# Autodesk Inventor assembly: CPRC16-6-6
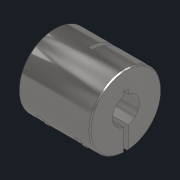
[picture p0: Inventor's stored thumbnail of the model, 180x180]
Saved by Autodesk Inventor 2022 (Build 260153000, 153)
## iProperties
Category: PARTsolutions
Company: MISUMI
Part Number: CPRC16-6-6
Catalog Web Link: www.cadenas.de
Description: CPRC, CPRSC-Couplings - Rigid - Clamping Type
Vendor: MISUMI
Document SubType Name: Assembly
Designer: partserver
Manufacturer: MISUMI
Mass: 2.52025 g
Surface Area: 21.4845 cm^2
Volume: 2.52025 cm^3
Density: 1 g/cm^3
PSOL_IDENT_0: {$CADENAS_DATA\23d-libs\misumi\metric\50_couplings\cprc_asmtab.prj},181 {VTYP=3D},{STYP=ASSTAB},{NB=
PSOL_IDENT_1: CPRC16-6-6},{LINA=CPRC16-6-6},{NN=CPRC, CPRSC},{DATE=30.06.2021 13:24:31},{GEOMDATE=17.01.2008},{VER
PSOL_IDENT_2: SION=},{LINEID=10},{WBVAR=MAT,DD1,DD2},{WBNUMERIC=}  {NB=CPRC16-6-6},{LINA=CPRC16-6-6},{KT=DUMMY},{P
PSOL_IDENT_3: N=CPRC16-6-6},{MAT=1},{MATALG='1','Aluminum Alloy','2','Stainless Steel'},{ST=Alumite},{AC=Hexagon S
PSOL_IDENT_4: ocket Head Cap Screws},{TYPE=CPRC},{D=16},{DD1=6},{DD1ALG1='5','5','6','6'},{DL=6},{DD2=6},{DD2ALG1='
PSOL_IDENT_5: 6','6'},{DR=6},{L=16},{M=2.5},{TSI=M2.5},{A=5},{A1=5.000},{TT=1},{TT1=1.000},{F=3.75},{T=1},{AT=0.3}
PSOL_IDENT_6: ,{F1=3.750},{TSI1=4.800},{SC1=2.500},{SC2=5.970},{TSMD=2.500},{TSMIN=2.013},{L6=4.000},{PPATH=cprc_t
PSOL_IDENT_7: emp.prj}
NB: CPRC16-6-6
NN: CPRC, CPRSC
NT: Couplings - Rigid - Clamping Type
NBSYN: $TYPE.$D.-$DD1.-$DD2.
LINA: CPRC16-6-6
CATALOG: Misumi
PN: CPRC16-6-6
MAT: Aluminum Alloy
ST: Clear Anodizing
AC: Hexagon Socket Head Cap Screws
D: 16
DD1: 6
DD2: 6
L: 16
M: 2.5
A: 5
TT: 1
F: 3.75
T: 1
SUPPLIER: MISUMI
ARTICLENO: CPRC16-6-6
BOMINFO: CPRC16-6-6
CREATOR: CADENAS GmbH
Title: CPRC16-6-6
Author: Cadenas PARTsolutions
Comments: Couplings - Rigid - Clamping Type
## Documents named in this file (3)
- C:\Users\yuta0\Downloads\0928\CPRC16-6-6.iam
- C:\Users\yuta0\Downloads\0928\D_CPRC16-6-6.ipt
- C:\Users\yuta0\Downloads\0928\M2_5.ipt
## Components (3 placed, 2 different names)
1. D_CPRC16-6-6:1 — L_XY@1 <-> SCW_XY@2, L_Z@1 <-> SCW_Z@2, L_YZ@1 <-> SCW_YZ@2, R_XY@1 <-> SCW_XY@3, R_Z@1 <-> SCW_Z@3, R_YZ@1 <-> SCW_YZ@3
2. M2_5:1 — L_XY@1 <-> SCW_XY@2, L_Z@1 <-> SCW_Z@2, L_YZ@1 <-> SCW_YZ@2
3. M2_5:2 — R_XY@1 <-> SCW_XY@3, R_Z@1 <-> SCW_Z@3, R_YZ@1 <-> SCW_YZ@3
## Relationships (6: Mate 4, Angle 2)
- L_XY@1 <-> SCW_XY@2 [Mate]: D_CPRC16-6-6:1 ↔ M2_5:1
- L_Z@1 <-> SCW_Z@2 [Mate]: D_CPRC16-6-6:1 ↔ M2_5:1
- L_YZ@1 <-> SCW_YZ@2 [Angle] (0 deg): D_CPRC16-6-6:1 ↔ M2_5:1
- R_XY@1 <-> SCW_XY@3 [Mate]: D_CPRC16-6-6:1 ↔ M2_5:2
- R_Z@1 <-> SCW_Z@3 [Mate]: D_CPRC16-6-6:1 ↔ M2_5:2
- R_YZ@1 <-> SCW_YZ@3 [Angle] (0 deg): D_CPRC16-6-6:1 ↔ M2_5:2
